# Autodesk Inventor assembly: 20_POL_Insert_Linear_Polarizer
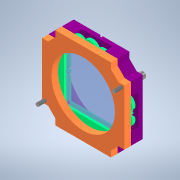
[picture p0: Inventor's stored thumbnail of the model, 180x180]
Saved by Autodesk Inventor 2022 (Build 260153000, 153)
## iProperties
Created: 2021-05-26
Part Number: 20_POL_Insert_Linear_Polarizer
Document SubType Name: Assembly
Designer: ASUS
Author: ASUS
## Documents named in this file (6)
- C:\Users\ASUS\Desktop\ASP - M.Sc. Photonics\Practical Modules\MODULE 3 - Research Project @IPHT-UC2\7.BUILD_ME\1.build_me_CADs\1. Crossed Polarizers\20_POL_Insert_Linear_Polarizer.iam
- C:\Users\ASUS\Desktop\ASP - M.Sc. Photonics\Practical Modules\MODULE 3 - Research Project @IPHT-UC2\7.BUILD_ME\1.build_me_CADs\1. Crossed Polarizers\20_POL_Insert_Linear_Polarizer_Guide.ipt
- C:\Users\ASUS\Desktop\ASP - M.Sc. Photonics\Practical Modules\MODULE 3 - Research Project @IPHT-UC2\7.BUILD_ME\1.build_me_CADs\1. Crossed Polarizers\20_POL_Insert_Linear_Polarizer_Lid.ipt
- C:\Users\ASUS\Desktop\ASP - M.Sc. Photonics\Practical Modules\MODULE 3 - Research Project @IPHT-UC2\7.BUILD_ME\1.build_me_CADs\1. Crossed Polarizers\20_POL_Insert_Linear_Polarizer_Wheel.ipt
- C:\Users\ASUS\Desktop\ASP - M.Sc. Photonics\Practical Modules\MODULE 3 - Research Project @IPHT-UC2\7.BUILD_ME\1.build_me_CADs\1. Crossed Polarizers\20_POL_Insert_Linear_Polarizer_Filter.ipt
- C:\Users\ASUS\Documents\Inventor\Content Center Files\R2022\en-US\DIN 912\DIN 912 - M2 x 0,4 x 16 x 15.ipt
## Components (6 placed, 5 different names)
1. 20_POL_Insert_Linear_Polarizer_Guide:1 — Rotational:5, Rotational:6
2. 20_POL_Insert_Linear_Polarizer_Lid:1 — Rigid:2, Rotational:7, Rotational:8
3. 20_POL_Insert_Linear_Polarizer_Wheel:1 — Rigid:1, Mate:1, Mate:2, Rotational:5, Rotational:6
4. 20_POL_Insert_Linear_Polarizer_Filter:1 — Rigid:1, Mate:1, Mate:2, Rigid:2
5. DIN 912 - replaced by DIN EN ISO 4762 M2 x 16:1 — Rotational:8
6. DIN 912 - replaced by DIN EN ISO 4762 M2 x 16:2 — Rotational:7
## Relationships (8: RevoluteJoint 4, WeldJoint 2, Mate 2)
- Rigid:1 [WeldJoint] (-1.5 mm): 20_POL_Insert_Linear_Polarizer_Wheel:1 ↔ 20_POL_Insert_Linear_Polarizer_Filter:1
- Mate:1: 20_POL_Insert_Linear_Polarizer_Wheel:1 ↔ 20_POL_Insert_Linear_Polarizer_Filter:1
- Mate:2: 20_POL_Insert_Linear_Polarizer_Wheel:1 ↔ 20_POL_Insert_Linear_Polarizer_Filter:1
- Rotational:5 [RevoluteJoint]: 20_POL_Insert_Linear_Polarizer_Guide:1 ↔ 20_POL_Insert_Linear_Polarizer_Wheel:1
- Rotational:6 [RevoluteJoint]: 20_POL_Insert_Linear_Polarizer_Guide:1 ↔ 20_POL_Insert_Linear_Polarizer_Wheel:1
- Rigid:2 [WeldJoint] (1.3 mm): 20_POL_Insert_Linear_Polarizer_Lid:1 ↔ 20_POL_Insert_Linear_Polarizer_Filter:1
- Rotational:7 [RevoluteJoint]: 20_POL_Insert_Linear_Polarizer_Lid:1 ↔ DIN 912 - replaced by DIN EN ISO 4762 M2 x 16:2
- Rotational:8 [RevoluteJoint]: 20_POL_Insert_Linear_Polarizer_Lid:1 ↔ DIN 912 - replaced by DIN EN ISO 4762 M2 x 16:1
